# Autodesk Inventor assembly: Rb PEEK
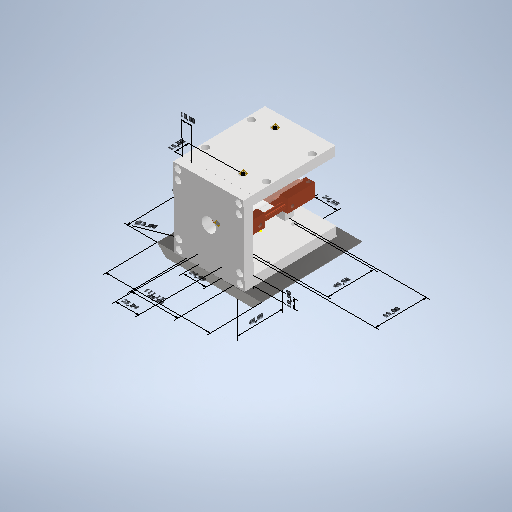
[picture p0: Inventor's stored thumbnail of the model, 512x512]
Saved by Autodesk Inventor 2025.3 (Build 293356000, 356)
## iProperties
Created: 2025-05-09
Part Number: Rb PEEK
Document SubType Name: Assembly
Designer: E. Moreno
Author: E. Moreno
Title: Rb PEEK - Ensamblado
## Documents named in this file (22)
- E:\Users\USER\Documents\GitHub\LAFriOC\Rb oven\Rb PEEK\Rb Full.iam
- E:\Users\USER\Documents\GitHub\LAFriOC\Rb oven\Rb PEEK\Rb PEEK - Arriba.ipt
- E:\Users\USER\Documents\GitHub\LAFriOC\Rb oven\Rb PEEK\Rb PEEK - Largo.ipt
- E:\Users\USER\Documents\GitHub\LAFriOC\Rb oven\Rb PEEK\Rb PEEK - Corto.ipt
- E:\Users\USER\Documents\GitHub\LAFriOC\Rb oven\Rb PEEK\Rb PEEK - Soporte.ipt
- E:\Users\USER\Documents\GitHub\LAFriOC\Rb oven\Rb PEEK\Rb PEEK - Abajo.ipt
- E:\Users\USER\Documents\GitHub\LAFriOC\Rb oven\Rb components\Cell.ipt
- E:\Users\USER\Documents\Inventor\Content Center Files\R2025\en-US\AS 1420\AS 1420 - 1973 - M4 x 25.ipt
- E:\Users\USER\Documents\Inventor\Content Center Files\R2025\en-US\AS 1420\AS 1420 - 1973 - M4 x 12.ipt
- E:\Users\USER\Documents\GitHub\LAFriOC\Rb oven\MS-1L Shield\Shield.iam
- E:\Users\USER\Documents\GitHub\LAFriOC\Rb oven\Rb PEEK\Rb PEEK - Largo_MIR.ipt
- E:\Users\USER\Documents\GitHub\LAFriOC\Rb oven\Rb components\Thermistor.ipt
- E:\Users\USER\Documents\GitHub\LAFriOC\Rb oven\Rb housing\Rb oven housing - Bottom.iam
- E:\Users\USER\Documents\GitHub\LAFriOC\Rb oven\Rb housing\Rb oven housing - Top.iam
- E:\Users\USER\Documents\GitHub\LAFriOC\Rb oven\Rb components\Heater1-4.ipt
- E:\Users\USER\Documents\GitHub\LAFriOC\Rb oven\Rb PEEK\Rb PEEK - Corto_MIR1_MIR.ipt
- E:\Users\USER\Documents\GitHub\LAFriOC\Rb oven\Rb PEEK\Rb Full\AIP\Cable and Harness\Thermistor Cable 1.iam
- E:\Users\USER\Documents\GitHub\LAFriOC\Rb oven\Rb PEEK\Rb Full\AIP\Cable and Harness\Thermistor Cable-2.iam
- E:\Users\USER\Documents\GitHub\LAFriOC\Rb oven\Rb PEEK\Rb Full\AIP\Cable and Harness\Heater Cable 1.iam
- E:\Users\USER\Documents\GitHub\LAFriOC\Rb oven\Rb PEEK\Rb Full\AIP\Cable and Harness\Heater Cable 2.iam
- E:\Users\USER\Documents\Inventor\Content Center Files\R2025\en-US\AS 1420\AS 1420 - 1973 - M4 x 20.ipt
- E:\Users\USER\Documents\Inventor\Content Center Files\R2025\en-US\AS 1420\AS 1420 - 1973 - M3 x 14.ipt
## Components (54 placed, 21 different names)
1. Shield:1 [sub-assembly] — Mate:57
2. Thermistor Cable 1 [sub-assembly]
3. Thermistor Cable-2 [sub-assembly]
4. Heater Cable 1 [sub-assembly]
5. Heater Cable 2 [sub-assembly]
6. Rb PEEK - Corto_MIR1_MIR:1 — Mate:53, Mate:54, Insert:68, Insert:69, Insert:70, Insert:71, Insert:72, Insert:73, Insert:74, Insert:75
7. Rb PEEK - Arriba:1 — Mate:1, Mate:2, Mate:3, Insert:10, Insert:11, Insert:12, Insert:13, Mate:54, Mate:56
8. Rb PEEK - Abajo:1 — Mate:21, Mate:22, Mate:23, Mate:29, Mate:30, Insert:21, Insert:24, Insert:25, Insert:26, Mate:38, Mate:39, Mate:44, Mate:45, Insert:46, Insert:47, Insert:56, Insert:57, Insert:58, Insert:59, Mate:57
9. Rb PEEK - Largo:1 — Mate:1, Mate:2, Mate:3, Mate:21, Mate:22, Mate:23, Mate:53, Mate:55
10. Rb PEEK - Largo_MIR:1 — Mate:38, Mate:39
11. Rb PEEK - Corto:2 — Mate:55, Mate:56, Insert:60, Insert:61, Insert:62, Insert:63, Insert:64, Insert:65, Insert:66, Insert:67
12. Rb PEEK - Soporte:1 — Mate:29, Mate:45, Mate:46
13. Rb PEEK - Soporte:2 — Mate:30, Mate:44
14. Cell:1 — Mate:43
15. Rb oven housing - Top:1 [sub-assembly] — Insert:38, Insert:39, Insert:40, Insert:41, Mate:42
16. Rb oven housing - Bottom:1 [sub-assembly] — Insert:42, Insert:43, Mate:42, Mate:43, Mate:46
17. Thermistor:1 — Mate:47
18. Thermistor:2
19. Heater1-4:1 — Insert:43, Mate:47
20. Heater1-4:2 — Insert:42
21. AS 1420 - Metric M4 x 20:9 — Insert:60
22. AS 1420 - Metric M4 x 20:10 — Insert:61
23. AS 1420 - Metric M4 x 20:11 — Insert:62
24. AS 1420 - Metric M4 x 20:12 — Insert:63
25. AS 1420 - Metric M4 x 20:13 — Insert:64
26. AS 1420 - Metric M4 x 20:14 — Insert:65
27. AS 1420 - Metric M4 x 20:15 — Insert:66
28. AS 1420 - Metric M4 x 20:16 — Insert:67
29. AS 1420 - Metric M4 x 20:17 — Insert:68
30. AS 1420 - Metric M4 x 20:18 — Insert:69
31. AS 1420 - Metric M4 x 20:19 — Insert:70
32. AS 1420 - Metric M4 x 20:20 — Insert:71
33. AS 1420 - Metric M4 x 20:21 — Insert:72
34. AS 1420 - Metric M4 x 20:22 — Insert:73
35. AS 1420 - Metric M4 x 20:23 — Insert:74
36. AS 1420 - Metric M4 x 20:24 — Insert:75
37. AS 1420 - Metric M4 x 25:21 — Insert:38
38. AS 1420 - Metric M4 x 25:22 — Insert:39
39. AS 1420 - Metric M4 x 25:23 — Insert:40
40. AS 1420 - Metric M4 x 25:24 — Insert:41
41. AS 1420 - Metric M3 x 14:1 — Insert:56
42. AS 1420 - Metric M3 x 14:2 — Insert:57
43. AS 1420 - Metric M3 x 14:3 — Insert:58
44. AS 1420 - Metric M3 x 14:4 — Insert:59
45. AS 1420 - Metric M4 x 25:6 — Insert:10
46. AS 1420 - Metric M4 x 25:7 — Insert:11
47. AS 1420 - Metric M4 x 25:8 — Insert:12
48. AS 1420 - Metric M4 x 25:9 — Insert:13
49. AS 1420 - Metric M4 x 25:13 — Insert:21
50. AS 1420 - Metric M4 x 25:14 — Insert:24
51. AS 1420 - Metric M4 x 25:15 — Insert:25
52. AS 1420 - Metric M4 x 25:16 — Insert:26
53. AS 1420 - Metric M4 x 12:7 — Insert:46
54. AS 1420 - Metric M4 x 12:8 — Insert:47
## Relationships (57: Insert 36, Mate 21)
- Mate:1: Rb PEEK - Arriba:1 ↔ Rb PEEK - Largo:1
- Mate:2: Rb PEEK - Arriba:1 ↔ Rb PEEK - Largo:1
- Mate:3: Rb PEEK - Arriba:1 ↔ Rb PEEK - Largo:1
- Mate:21: Rb PEEK - Abajo:1 ↔ Rb PEEK - Largo:1
- Mate:22: Rb PEEK - Abajo:1 ↔ Rb PEEK - Largo:1
- Mate:23: Rb PEEK - Abajo:1 ↔ Rb PEEK - Largo:1
- Mate:29: Rb PEEK - Abajo:1 ↔ Rb PEEK - Soporte:1
- Mate:30: Rb PEEK - Abajo:1 ↔ Rb PEEK - Soporte:2
- Insert:10: Rb PEEK - Arriba:1 ↔ AS 1420 - Metric M4 x 25:6
- Insert:11: Rb PEEK - Arriba:1 ↔ AS 1420 - Metric M4 x 25:7
- Insert:12: Rb PEEK - Arriba:1 ↔ AS 1420 - Metric M4 x 25:8
- Insert:13: Rb PEEK - Arriba:1 ↔ AS 1420 - Metric M4 x 25:9
- Insert:21: Rb PEEK - Abajo:1 ↔ AS 1420 - Metric M4 x 25:13
- Insert:24: Rb PEEK - Abajo:1 ↔ AS 1420 - Metric M4 x 25:14
- Insert:25: Rb PEEK - Abajo:1 ↔ AS 1420 - Metric M4 x 25:15
- Insert:26: Rb PEEK - Abajo:1 ↔ AS 1420 - Metric M4 x 25:16
- Mate:38: Rb PEEK - Abajo:1 ↔ Rb PEEK - Largo_MIR:1
- Mate:39: Rb PEEK - Abajo:1 ↔ Rb PEEK - Largo_MIR:1
- Insert:38: Rb oven housing - Top:1 ↔ AS 1420 - Metric M4 x 25:21
- Insert:39: Rb oven housing - Top:1 ↔ AS 1420 - Metric M4 x 25:22
- Insert:40: Rb oven housing - Top:1 ↔ AS 1420 - Metric M4 x 25:23
- Insert:41: Rb oven housing - Top:1 ↔ AS 1420 - Metric M4 x 25:24
- Insert:42 (-10.5 mm): Rb oven housing - Bottom:1 ↔ Heater1-4:2
- Insert:43 (-10.5 mm): Rb oven housing - Bottom:1 ↔ Heater1-4:1
- Mate:42: Rb oven housing - Top:1 ↔ Rb oven housing - Bottom:1
- Mate:43: Cell:1 ↔ Rb oven housing - Bottom:1
- Mate:44: Rb PEEK - Abajo:1 ↔ Rb PEEK - Soporte:2
- Mate:45: Rb PEEK - Abajo:1 ↔ Rb PEEK - Soporte:1
- Insert:46: Rb PEEK - Abajo:1 ↔ AS 1420 - Metric M4 x 12:7
- Insert:47: Rb PEEK - Abajo:1 ↔ AS 1420 - Metric M4 x 12:8
- Mate:46: Rb PEEK - Soporte:1 ↔ Rb oven housing - Bottom:1
- Mate:47 (-4.3 mm): Thermistor:1 ↔ Heater1-4:1
- Mate:53: Rb PEEK - Corto_MIR1_MIR:1 ↔ Rb PEEK - Largo:1
- Mate:54: Rb PEEK - Corto_MIR1_MIR:1 ↔ Rb PEEK - Arriba:1
- Mate:55: Rb PEEK - Largo:1 ↔ Rb PEEK - Corto:2
- Mate:56: Rb PEEK - Arriba:1 ↔ Rb PEEK - Corto:2
- Insert:56: Rb PEEK - Abajo:1 ↔ AS 1420 - Metric M3 x 14:1
- Insert:57: Rb PEEK - Abajo:1 ↔ AS 1420 - Metric M3 x 14:2
- Insert:58: Rb PEEK - Abajo:1 ↔ AS 1420 - Metric M3 x 14:3
- Insert:59: Rb PEEK - Abajo:1 ↔ AS 1420 - Metric M3 x 14:4
- Mate:57: Shield:1 ↔ Rb PEEK - Abajo:1
- Insert:60: Rb PEEK - Corto:2 ↔ AS 1420 - Metric M4 x 20:9
- Insert:61: Rb PEEK - Corto:2 ↔ AS 1420 - Metric M4 x 20:10
- Insert:62: Rb PEEK - Corto:2 ↔ AS 1420 - Metric M4 x 20:11
- Insert:63: Rb PEEK - Corto:2 ↔ AS 1420 - Metric M4 x 20:12
- Insert:64: Rb PEEK - Corto:2 ↔ AS 1420 - Metric M4 x 20:13
- Insert:65: Rb PEEK - Corto:2 ↔ AS 1420 - Metric M4 x 20:14
- Insert:66: Rb PEEK - Corto:2 ↔ AS 1420 - Metric M4 x 20:15
- Insert:67: Rb PEEK - Corto:2 ↔ AS 1420 - Metric M4 x 20:16
- Insert:68: Rb PEEK - Corto_MIR1_MIR:1 ↔ AS 1420 - Metric M4 x 20:17
- Insert:69: Rb PEEK - Corto_MIR1_MIR:1 ↔ AS 1420 - Metric M4 x 20:18
- Insert:70: Rb PEEK - Corto_MIR1_MIR:1 ↔ AS 1420 - Metric M4 x 20:19
- Insert:71: Rb PEEK - Corto_MIR1_MIR:1 ↔ AS 1420 - Metric M4 x 20:20
- Insert:72: Rb PEEK - Corto_MIR1_MIR:1 ↔ AS 1420 - Metric M4 x 20:21
- Insert:73: Rb PEEK - Corto_MIR1_MIR:1 ↔ AS 1420 - Metric M4 x 20:22
- Insert:74: Rb PEEK - Corto_MIR1_MIR:1 ↔ AS 1420 - Metric M4 x 20:23
- Insert:75: Rb PEEK - Corto_MIR1_MIR:1 ↔ AS 1420 - Metric M4 x 20:24
